# Autodesk Inventor assembly: ttp lmp
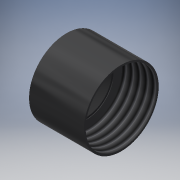
[picture p0: Inventor's stored thumbnail of the model, 180x180]
Saved by Autodesk Inventor 2019.5 (Build 235369000, 369)
## iProperties
Created: 2022-10-11
Part Number: ttp lmp
Document SubType Name: Assembly
Designer: ASUS
Author: ASUS
## Documents named in this file (3)
- C:\Users\ASUS\Downloads\produk fri-074\ttp lmp.iam
- C:\Users\ASUS\Downloads\produk fri-074\Tutup lampu.ipt
- C:\Users\ASUS\Downloads\produk fri-074\gabung sama tutup lampu.ipt
## Components (2 placed, 2 different names)
1. Tutup lampu:1 — Mate:1
2. gabung sama tutup lampu:1 — Mate:1
## Relationships (1: Mate 1)
- Mate:1: Tutup lampu:1 ↔ gabung sama tutup lampu:1
